# Autodesk Inventor assembly: Trappe Lancement
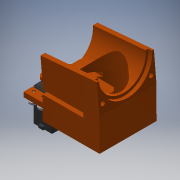
[picture p0: Inventor's stored thumbnail of the model, 180x180]
Saved by Autodesk Inventor 2016 SP1 (Build 200210100, 210)
## iProperties
Created: 2017-04-26
Part Number: Trappe Lancement
Material: Générique
Document SubType Name: Assembly
Designer: dimercur
Author: dimercur
## Documents named in this file (6)
- D:\Users\dimercur\Documents\git\dev-gei\dev-gei2\Circuit-a-Bille\Trappe Lancement.iam
- D:\Users\dimercur\Documents\git\dev-gei\dev-gei2\Circuit-a-Bille\Trappe lancement.ipt
- D:\Users\dimercur\Documents\git\dev-gei\dev-gei2\Circuit-a-Bille\Pieces importées\Futaba-s3004.ipt
- D:\Users\dimercur\Documents\Inventor\Content Center Files\R2016\fr-FR\AS B194 PR2 AB\AS B194 - N° 10 x 5_16-PR2 AB.ipt
- D:\Users\dimercur\Documents\git\dev-gei\dev-gei2\Circuit-a-Bille\Loquet Lancement.ipt
- D:\Users\dimercur\Documents\Inventor\Content Center Files\R2016\fr-FR\AS B194 PR2 AB\AS B194 - N° 2 x 1_8-PR2 AB.ipt
## Components (8 placed, 5 different names)
1. Trappe lancement:1 — Placage:2, Cylindrique:1, Placage:3
2. Futaba-s3004:1 — Placage:2, Cylindrique:1, Placage:3, Logement:1, Logement:2, Logement:3, Logement:4, Placage:4, Cylindrique:2
3. AS B194 PR2 AB N° 10 x 5/16-PR2 AB:1 — Logement:1
4. AS B194 PR2 AB N° 10 x 5/16-PR2 AB:2 — Logement:2
5. AS B194 PR2 AB N° 10 x 5/16-PR2 AB:3 — Logement:3
6. AS B194 PR2 AB N° 10 x 5/16-PR2 AB:4 — Logement:4
7. Loquet Lancement:1 — Placage:4, Cylindrique:2, Logement:5
8. AS B194 PR2 AB N° 2 x 1/8-PR2 AB:1 — Logement:5
## Relationships (10: Insert 5, Mate 3, CylindricalJoint 2)
- Placage:2 [Mate]: Trappe lancement:1 ↔ Futaba-s3004:1
- Cylindrique:1: Trappe lancement:1 ↔ Futaba-s3004:1
- Placage:3 [Mate]: Trappe lancement:1 ↔ Futaba-s3004:1
- Logement:1 [Insert]: Futaba-s3004:1 ↔ AS B194 PR2 AB N° 10 x 5/16-PR2 AB:1
- Logement:2 [Insert]: Futaba-s3004:1 ↔ AS B194 PR2 AB N° 10 x 5/16-PR2 AB:2
- Logement:3 [Insert]: Futaba-s3004:1 ↔ AS B194 PR2 AB N° 10 x 5/16-PR2 AB:3
- Logement:4 [Insert]: Futaba-s3004:1 ↔ AS B194 PR2 AB N° 10 x 5/16-PR2 AB:4
- Placage:4 [Mate]: Futaba-s3004:1 ↔ Loquet Lancement:1
- Cylindrique:2: Futaba-s3004:1 ↔ Loquet Lancement:1
- Logement:5 [Insert]: Loquet Lancement:1 ↔ AS B194 PR2 AB N° 2 x 1/8-PR2 AB:1
